# Autodesk Inventor assembly: full_instalation
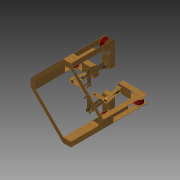
[picture p0: Inventor's stored thumbnail of the model, 180x180]
Saved by Autodesk Inventor 2013 (Build 170138000, 138)
## iProperties
Created: 2014-10-20
Part Number: full_instalation
Document SubType Name: Assembly
Designer: Masta
Author: Masta
## Documents named in this file (2)
- D:\DrOctopus\3D model\full_instalation.iam
- D:\DrOctopus\3D model\one_unit.iam
## Components (4 placed, 1 different names)
1. one_unit:1 [sub-assembly] — Flush:1, Flush:2, Flush:3, Mate:1, Flush:4, Mate:2, Flush:5
2. one_unit:2 [sub-assembly] — Flush:1, Mate:3, Flush:6
3. one_unit:3 [sub-assembly] — Flush:3, Mate:2, Flush:5
4. one_unit:4 [sub-assembly] — Flush:2, Mate:1, Flush:4, Mate:3, Flush:6
## Relationships (9: Flush 6, Mate 3)
- Flush:1: one_unit:1 ↔ one_unit:2
- Flush:2: one_unit:1 ↔ one_unit:4
- Flush:3: one_unit:1 ↔ one_unit:3
- Mate:1: one_unit:1 ↔ one_unit:4
- Flush:4: one_unit:1 ↔ one_unit:4
- Mate:2: one_unit:1 ↔ one_unit:3
- Flush:5: one_unit:1 ↔ one_unit:3
- Mate:3: one_unit:2 ↔ one_unit:4
- Flush:6: one_unit:2 ↔ one_unit:4
